# Autodesk Inventor assembly: BaseEnsamble
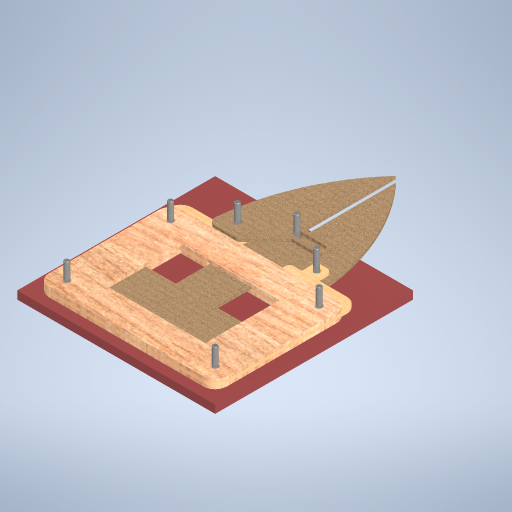
[picture p0: Inventor's stored thumbnail of the model, 512x512]
Saved by Autodesk Inventor 2023.1 (Build 271208000, 208)
## iProperties
Created: 2022-11-11
Part Number: BaseEnsamble
Document SubType Name: Assembly
Designer: Daniel Peña
Author: Daniel Peña
## Documents named in this file (5)
- E:\Daniel DiscoA\Documents\UNAL\ProyectoRobotica\CAD\V3 - BigChungus\BaseEnsamble.iam
- E:\Daniel DiscoA\Documents\UNAL\ProyectoRobotica\CAD\V3 - BigChungus\Piso.ipt
- E:\Daniel DiscoA\Documents\UNAL\ProyectoRobotica\CAD\V3 - BigChungus\Gripper General.iam
- E:\Daniel DiscoA\Documents\UNAL\ProyectoRobotica\CAD\V3 - BigChungus\PortaTornillos.ipt
- E:\Daniel DiscoA\Documents\Inventor\Content Center Files\R2023\en-US\AS 1420\AS 1420 - 1973 - M5 x 25.ipt
## Components (10 placed, 4 different names)
1. Piso:1 — Flush:1
2. Gripper General:1 [sub-assembly] — Mate:1, Flush:2, Flush:3
3. PortaTornillos:1 — Flush:1, Mate:1, Flush:2, Flush:3, Insert:1, Insert:2, Insert:3, Insert:4, Insert:5, Insert:6, Insert:7
4. AS 1420 - Metric M5 x 25:1 — Insert:2
5. AS 1420 - Metric M5 x 25:2 — Insert:1
6. AS 1420 - Metric M5 x 25:3 — Insert:3
7. AS 1420 - Metric M5 x 25:4 — Insert:5
8. AS 1420 - Metric M5 x 25:5 — Insert:4
9. AS 1420 - Metric M5 x 25:6 — Insert:6
10. AS 1420 - Metric M5 x 25:7 — Insert:7
## Relationships (11: Insert 7, Flush 3, Mate 1)
- Flush:1: Piso:1 ↔ PortaTornillos:1
- Mate:1: Gripper General:1 ↔ PortaTornillos:1
- Flush:2 (10 mm): Gripper General:1 ↔ PortaTornillos:1
- Flush:3 (-10 mm): Gripper General:1 ↔ PortaTornillos:1
- Insert:1: PortaTornillos:1 ↔ AS 1420 - Metric M5 x 25:2
- Insert:2: PortaTornillos:1 ↔ AS 1420 - Metric M5 x 25:1
- Insert:3: PortaTornillos:1 ↔ AS 1420 - Metric M5 x 25:3
- Insert:4: PortaTornillos:1 ↔ AS 1420 - Metric M5 x 25:5
- Insert:5: PortaTornillos:1 ↔ AS 1420 - Metric M5 x 25:4
- Insert:6: PortaTornillos:1 ↔ AS 1420 - Metric M5 x 25:6
- Insert:7: PortaTornillos:1 ↔ AS 1420 - Metric M5 x 25:7
